# Autodesk Inventor assembly: единое крепление
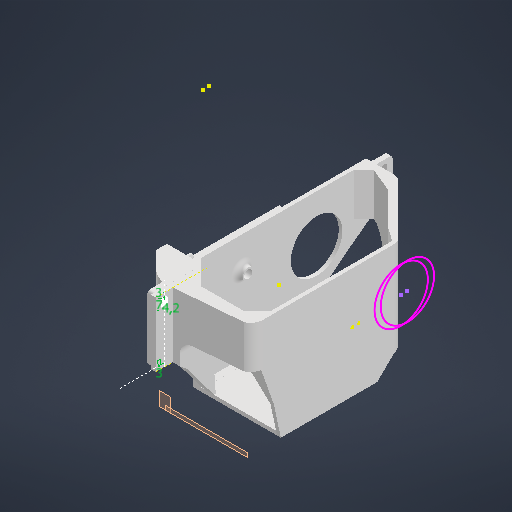
[picture p0: Inventor's stored thumbnail of the model, 512x512]
Saved by Autodesk Inventor 2025 (Build 290162000, 162)
## iProperties
Created: 2024-09-25
Part Number: единое крепление
Document SubType Name: Assembly
Designer: GameHD
Author: GameHD
## Documents named in this file (5)
- C:\Users\GameHD\Desktop\что-то нужное\Phantom16950\единое крепление.iam
- C:\Users\GameHD\Desktop\что-то нужное\Phantom16950\крепл для колёс.ipt
- C:\Users\GameHD\Desktop\что-то нужное\Phantom16950\крепл для колёс. 2 часть.ipt
- C:\Users\GameHD\Desktop\что-то нужное\Phantom16950\крепл для колёс встав часть. вторая часть.ipt
- C:\Users\GameHD\Desktop\что-то нужное\Phantom16950\крепл для колёс встав часть.ipt
## Components (4 placed, 4 different names)
1. крепл для колёс:1 — Совмещение:4, Заподлицо:5, Совмещение:5, Заподлицо:7
2. крепл для колёс. 2 часть:1 — Совмещение:4, Заподлицо:5, Совмещение:6, Заподлицо:8
3. крепл для колёс встав часть. вторая часть:1 — Совмещение:6, Заподлицо:6, Совмещение:7, Заподлицо:7, Заподлицо:8
4. крепл для колёс встав часть:1 — Совмещение:5, Заподлицо:6, Совмещение:7
## Relationships (8: Mate 4, Flush 4)
- Совмещение:4 [Mate]: крепл для колёс:1 ↔ крепл для колёс. 2 часть:1
- Заподлицо:5 [Flush]: крепл для колёс:1 ↔ крепл для колёс. 2 часть:1
- Совмещение:5 [Mate]: крепл для колёс:1 ↔ крепл для колёс встав часть:1
- Совмещение:6 [Mate]: крепл для колёс. 2 часть:1 ↔ крепл для колёс встав часть. вторая часть:1
- Заподлицо:6 [Flush]: крепл для колёс встав часть. вторая часть:1 ↔ крепл для колёс встав часть:1
- Совмещение:7 [Mate]: крепл для колёс встав часть. вторая часть:1 ↔ крепл для колёс встав часть:1
- Заподлицо:7 [Flush]: крепл для колёс:1 ↔ крепл для колёс встав часть. вторая часть:1
- Заподлицо:8 [Flush]: крепл для колёс. 2 часть:1 ↔ крепл для колёс встав часть. вторая часть:1
